# Autodesk Inventor assembly: Craftsman Socket U-Joint_4
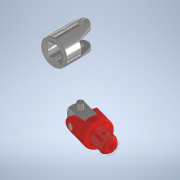
[picture p0: Inventor's stored thumbnail of the model, 180x180]
Saved by Autodesk Inventor 2021 (Build 250183000, 183)
## iProperties
Created: 2013-08-30
Part Number: Craftsman Socket U-Joint_4
Document SubType Name: Assembly
Designer: techv
Author: techv
## Documents named in this file (4)
- D:\Projects\P_Borewell\V2\Design\Craftsman Socket U-Joint_4.iam
- D:\Projects\P_Borewell\V2\Design\Craftsman Socket U-Joint Base.ipt
- D:\Projects\P_Borewell\V2\Design\Craftsman Socket U-Joint Intermediate Body.ipt
- D:\Projects\P_Borewell\V2\Design\Craftsman Socket U-Joint Drive.ipt
## Components (3 placed, 3 different names)
1. Craftsman Socket U-Joint Base:1 — Mate:3
2. Craftsman Socket U-Joint Intermediate Body:1 — Mate:1, Mate:2, Mate:3, Mate:4, Mate:5
3. Craftsman Socket U-Joint Drive:1 — Mate:1, Mate:2, Mate:4, Mate:5
## Relationships (5: Mate 5)
- Mate:1: Craftsman Socket U-Joint Intermediate Body:1 ↔ Craftsman Socket U-Joint Drive:1
- Mate:2: Craftsman Socket U-Joint Intermediate Body:1 ↔ Craftsman Socket U-Joint Drive:1
- Mate:3: Craftsman Socket U-Joint Base:1 ↔ Craftsman Socket U-Joint Intermediate Body:1
- Mate:4: Craftsman Socket U-Joint Intermediate Body:1 ↔ Craftsman Socket U-Joint Drive:1
- Mate:5: Craftsman Socket U-Joint Intermediate Body:1 ↔ Craftsman Socket U-Joint Drive:1
